# Autodesk Inventor assembly: Weapon Assembly
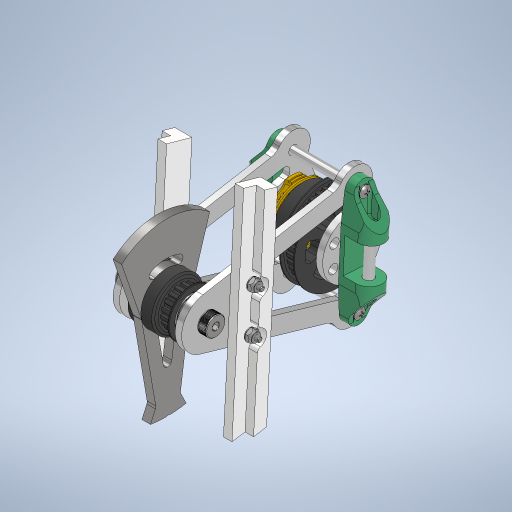
[picture p0: Inventor's stored thumbnail of the model, 512x512]
Saved by Autodesk Inventor 2023.2 (Build 272271000, 271)
## iProperties
Created: 2022-05-21
Part Number: Weapon Assembly
Document SubType Name: Assembly
Designer: Nathan Cai
Mass: 625.577 g
Surface Area: 1409.18 cm^2
Volume: 227.374 cm^3
Density: 2.75131 g/cm^3
Author: Nathan Cai
## Documents named in this file (14)
- E:\Documents\Inventor\0.3rd Lawette - V3.5\Vertical Weapon Assembly (3rd Law)\Weapon Assembly (3rd Law).iam
- E:\Documents\Inventor\0.3rd Lawette - V3.5\Standoff 1.5in.ipt
- E:\Documents\Inventor\Content Center Files\R2023\en-US\ANSI B18.6.3(27)\ANSI B18.6.3 - 6-32 UNC - 0.75(11).ipt
- E:\Documents\Inventor\Content Center Files\R2023\en-US\SAE J773b\SAE J773b - No. 6. SAE Type L. narrow.ipt
- E:\Documents\Inventor\Content Center Files\R2023\en-US\IFI 100 107(2)\IFI 100_107 - No. 6 - 32 Metal Type.ipt
- E:\Documents\Inventor\0.3rd Lawette - V3.5\Bracket.ipt
- E:\Documents\Inventor\Content Center Files\R2023\en-US\ANSI B18.6.3(27)\ANSI B18.6.3 - 6-32 UNC - 0.625(11).ipt
- E:\Documents\Inventor\0.3rd Lawette - V3.5\Vertical Weapon Assembly (3rd Law)\Legs.ipt
- E:\Documents\Inventor\0.3rd Lawette - V3.5\Vertical Weapon Assembly (3rd Law)\Frame (Motor Side).ipt
- E:\Documents\Inventor\0.3rd Lawette - V3.5\Vertical Weapon Assembly (3rd Law)\90630A121_High-Strength Steel Nylon-Insert Locknut.ipt
- E:\Documents\Inventor\0.3rd Lawette - V3.5\Vertical Weapon Assembly (3rd Law)\90807A139_Same-Size Thread Alloy Steel Shoulder Screw.ipt
- E:\Documents\Inventor\0.3rd Lawette - V3.5\Vertical Weapon Assembly (3rd Law)\Weapon (Motor-Side Pulley).iam
- E:\Documents\Inventor\0.3rd Lawette - V3.5\Vertical Weapon Assembly (3rd Law)\Weapon (Weapon-Side Pulley).iam
- E:\Documents\Inventor\0.3rd Lawette - V3.5\Standoff 2in.ipt
## Components (42 placed, 13 different names)
1. Weapon (Weapon-Side Pulley):2 [sub-assembly]
2. Weapon (Motor-Side Pulley):2 [sub-assembly] — Mate:249
3. 90807A139_Same-Size Thread Alloy Steel Shoulder Screw:2
4. 90630A121_High-Strength Steel Nylon-Insert Locknut:2
5. Frame (Motor Side):2 — Mate:245, Mate:249
6. Frame (Motor Side):3 — Mate:234, Mate:235, Mate:236, Mate:237, Mate:238, Mate:239, Mate:240, Mate:242, Mate:247
7. Legs:3 — Mate:234, Mate:235, Mate:241, Mate:243
8. Legs:2 — Mate:231, Mate:233
9. Bracket:1 — Mate:176, Flush:2, Mate:210, Mate:211, Mate:212, Mate:213, Mate:218, Mate:219, Mate:221, Mate:222, Mate:244, Mate:246, Mate:248
10. Bracket:2 — Mate:177, Flush:1, Mate:214, Mate:215, Mate:216, Mate:217, Mate:220, Mate:224, Mate:244
11. Standoff 1.5in:3 — Mate:176, Flush:2, Mate:223, Mate:225
12. Standoff 1.5in:4 — Mate:177, Flush:1
13. Cross Recessed Truss Head Machine Screw - Type I - Inch No. 6 - 32 - 3/4:29 — Mate:236, Mate:237
14. Conical Spring Washer SAE J773b (Inch) No. 6. SAE Type L. narrow:40 — Mate:240, Mate:241, Insert:47
15. Prevailing Torque Type Hex Nut - Inch (IFI) No. 6 - 32 Metal Type:24 — Insert:47
16. Cross Recessed Truss Head Machine Screw - Type I - Inch No. 6 - 32 - 3/4:30 — Mate:238, Mate:239
17. Conical Spring Washer SAE J773b (Inch) No. 6. SAE Type L. narrow:41 — Mate:242, Mate:243, Insert:48
18. Prevailing Torque Type Hex Nut - Inch (IFI) No. 6 - 32 Metal Type:25 — Insert:48
19. Standoff 2in:1 — Mate:245, Mate:246
20. Standoff 2in:2 — Mate:247, Mate:248
21. Prevailing Torque Type Hex Nut - Inch (IFI) No. 6 - 32 Metal Type:23 — Insert:46
22. Conical Spring Washer SAE J773b (Inch) No. 6. SAE Type L. narrow:39 — Mate:233, Insert:46
23. Cross Recessed Truss Head Machine Screw - Type I - Inch No. 6 - 32 - 3/4:28
24. Prevailing Torque Type Hex Nut - Inch (IFI) No. 6 - 32 Metal Type:19 — Insert:45
25. Conical Spring Washer SAE J773b (Inch) No. 6. SAE Type L. narrow:27 — Mate:231, Insert:45
26. Cross Recessed Truss Head Machine Screw - Type I - Inch No. 6 - 32 - 3/4:20
27. Cross Recessed Truss Head Machine Screw - Type I - Inch No. 6 - 32 - 5/8:8 — Insert:44
28. Conical Spring Washer SAE J773b (Inch) No. 6. SAE Type L. narrow:38 — Mate:224, Mate:225, Insert:44
29. Cross Recessed Truss Head Machine Screw - Type I - Inch No. 6 - 32 - 5/8:7 — Insert:43
30. Conical Spring Washer SAE J773b (Inch) No. 6. SAE Type L. narrow:37 — Mate:222, Mate:223, Insert:43
31. Cross Recessed Truss Head Machine Screw - Type I - Inch No. 6 - 32 - 5/8:6 — Insert:42
32. Conical Spring Washer SAE J773b (Inch) No. 6. SAE Type L. narrow:36 — Mate:220, Mate:221, Insert:42
33. Cross Recessed Truss Head Machine Screw - Type I - Inch No. 6 - 32 - 5/8:5 — Insert:41
34. Conical Spring Washer SAE J773b (Inch) No. 6. SAE Type L. narrow:35 — Mate:218, Mate:219, Insert:41
35. Cross Recessed Truss Head Machine Screw - Type I - Inch No. 6 - 32 - 3/4:27 — Insert:40
36. Conical Spring Washer SAE J773b (Inch) No. 6. SAE Type L. narrow:34 — Mate:216, Mate:217, Insert:40
37. Cross Recessed Truss Head Machine Screw - Type I - Inch No. 6 - 32 - 3/4:26 — Insert:39
38. Conical Spring Washer SAE J773b (Inch) No. 6. SAE Type L. narrow:33 — Mate:214, Mate:215, Insert:39
39. Cross Recessed Truss Head Machine Screw - Type I - Inch No. 6 - 32 - 3/4:25 — Insert:38
40. Conical Spring Washer SAE J773b (Inch) No. 6. SAE Type L. narrow:32 — Mate:212, Mate:213, Insert:38
41. Cross Recessed Truss Head Machine Screw - Type I - Inch No. 6 - 32 - 3/4:24 — Insert:37
42. Conical Spring Washer SAE J773b (Inch) No. 6. SAE Type L. narrow:31 — Mate:210, Mate:211, Insert:37
## Relationships (73: Mate 58, Insert 12, Flush 2, Symmetry 1)
- [Mate]: 90807A139_Same-Size Thread Alloy Steel Shoulder Screw:2 ↔ 90630A121_High-Strength Steel Nylon-Insert Locknut:2
- [Mate] (50.8 mm): 90807A139_Same-Size Thread Alloy Steel Shoulder Screw:2 ↔ 90630A121_High-Strength Steel Nylon-Insert Locknut:2
- [Mate]: Weapon (Weapon-Side Pulley):2 ↔ 90807A139_Same-Size Thread Alloy Steel Shoulder Screw:2
- [Mate]: 90807A139_Same-Size Thread Alloy Steel Shoulder Screw:2 ↔ Frame (Motor Side):2
- [Mate]: 90807A139_Same-Size Thread Alloy Steel Shoulder Screw:2 ↔ Frame (Motor Side):3
- [Mate]: 90807A139_Same-Size Thread Alloy Steel Shoulder Screw:2 ↔ Frame (Motor Side):3
- [Mate]: Frame (Motor Side):2 ↔ Frame (Motor Side):3
- [Mate]: Frame (Motor Side):3 ↔ Legs:3
- [Mate] (0.0254 mm): Weapon (Weapon-Side Pulley):2 ↔ Frame (Motor Side):2
- [Symmetry]: Frame (Motor Side):2 ↔ Frame (Motor Side):3
- [Mate]: Frame (Motor Side):2 ↔ Legs:2
- [Mate]: Frame (Motor Side):2 ↔ Legs:2
- [Mate]: Frame (Motor Side):2 ↔ Legs:2
- [Mate]: Weapon (Motor-Side Pulley):2 ↔ Frame (Motor Side):2
- [Mate]: Weapon (Motor-Side Pulley):2 ↔ Frame (Motor Side):2
- [Mate]: Frame (Motor Side):2 ↔ Bracket:2
- [Mate]: Frame (Motor Side):3 ↔ Bracket:1
- Mate:176: Bracket:1 ↔ Standoff 1.5in:3
- Mate:177: Bracket:2 ↔ Standoff 1.5in:4
- Flush:1: Bracket:2 ↔ Standoff 1.5in:4
- Flush:2: Bracket:1 ↔ Standoff 1.5in:3
- Mate:210: Bracket:1 ↔ Conical Spring Washer SAE J773b (Inch) No. 6. SAE Type L. narrow:31
- Mate:211: Bracket:1 ↔ Conical Spring Washer SAE J773b (Inch) No. 6. SAE Type L. narrow:31
- Mate:212: Bracket:1 ↔ Conical Spring Washer SAE J773b (Inch) No. 6. SAE Type L. narrow:32
- Mate:213: Bracket:1 ↔ Conical Spring Washer SAE J773b (Inch) No. 6. SAE Type L. narrow:32
- Insert:37: Cross Recessed Truss Head Machine Screw - Type I - Inch No. 6 - 32 - 3/4:24 ↔ Conical Spring Washer SAE J773b (Inch) No. 6. SAE Type L. narrow:31
- Insert:38: Cross Recessed Truss Head Machine Screw - Type I - Inch No. 6 - 32 - 3/4:25 ↔ Conical Spring Washer SAE J773b (Inch) No. 6. SAE Type L. narrow:32
- Mate:214: Bracket:2 ↔ Conical Spring Washer SAE J773b (Inch) No. 6. SAE Type L. narrow:33
- Mate:215: Bracket:2 ↔ Conical Spring Washer SAE J773b (Inch) No. 6. SAE Type L. narrow:33
- Mate:216: Bracket:2 ↔ Conical Spring Washer SAE J773b (Inch) No. 6. SAE Type L. narrow:34
- Mate:217: Bracket:2 ↔ Conical Spring Washer SAE J773b (Inch) No. 6. SAE Type L. narrow:34
- Insert:39: Cross Recessed Truss Head Machine Screw - Type I - Inch No. 6 - 32 - 3/4:26 ↔ Conical Spring Washer SAE J773b (Inch) No. 6. SAE Type L. narrow:33
- Insert:40: Cross Recessed Truss Head Machine Screw - Type I - Inch No. 6 - 32 - 3/4:27 ↔ Conical Spring Washer SAE J773b (Inch) No. 6. SAE Type L. narrow:34
- Mate:218: Bracket:1 ↔ Conical Spring Washer SAE J773b (Inch) No. 6. SAE Type L. narrow:35
- Mate:219: Bracket:1 ↔ Conical Spring Washer SAE J773b (Inch) No. 6. SAE Type L. narrow:35
- Mate:220: Bracket:2 ↔ Conical Spring Washer SAE J773b (Inch) No. 6. SAE Type L. narrow:36
- Mate:221: Bracket:1 ↔ Conical Spring Washer SAE J773b (Inch) No. 6. SAE Type L. narrow:36
- Insert:41: Cross Recessed Truss Head Machine Screw - Type I - Inch No. 6 - 32 - 5/8:5 ↔ Conical Spring Washer SAE J773b (Inch) No. 6. SAE Type L. narrow:35
- Insert:42: Cross Recessed Truss Head Machine Screw - Type I - Inch No. 6 - 32 - 5/8:6 ↔ Conical Spring Washer SAE J773b (Inch) No. 6. SAE Type L. narrow:36
- Mate:222: Bracket:1 ↔ Conical Spring Washer SAE J773b (Inch) No. 6. SAE Type L. narrow:37
- Mate:223: Standoff 1.5in:3 ↔ Conical Spring Washer SAE J773b (Inch) No. 6. SAE Type L. narrow:37
- Mate:224: Bracket:2 ↔ Conical Spring Washer SAE J773b (Inch) No. 6. SAE Type L. narrow:38
- Mate:225: Standoff 1.5in:3 ↔ Conical Spring Washer SAE J773b (Inch) No. 6. SAE Type L. narrow:38
- Insert:43: Cross Recessed Truss Head Machine Screw - Type I - Inch No. 6 - 32 - 5/8:7 ↔ Conical Spring Washer SAE J773b (Inch) No. 6. SAE Type L. narrow:37
- Insert:44: Cross Recessed Truss Head Machine Screw - Type I - Inch No. 6 - 32 - 5/8:8 ↔ Conical Spring Washer SAE J773b (Inch) No. 6. SAE Type L. narrow:38
- [Mate]: Frame (Motor Side):2 ↔ Cross Recessed Truss Head Machine Screw - Type I - Inch No. 6 - 32 - 3/4:20
- [Mate]: Frame (Motor Side):2 ↔ Cross Recessed Truss Head Machine Screw - Type I - Inch No. 6 - 32 - 3/4:20
- [Mate]: Frame (Motor Side):2 ↔ Cross Recessed Truss Head Machine Screw - Type I - Inch No. 6 - 32 - 3/4:28
- [Mate]: Frame (Motor Side):2 ↔ Cross Recessed Truss Head Machine Screw - Type I - Inch No. 6 - 32 - 3/4:28
- [Mate]: Frame (Motor Side):2 ↔ Conical Spring Washer SAE J773b (Inch) No. 6. SAE Type L. narrow:27
- Mate:231: Legs:2 ↔ Conical Spring Washer SAE J773b (Inch) No. 6. SAE Type L. narrow:27
- [Mate]: Frame (Motor Side):2 ↔ Conical Spring Washer SAE J773b (Inch) No. 6. SAE Type L. narrow:39
- Mate:233: Legs:2 ↔ Conical Spring Washer SAE J773b (Inch) No. 6. SAE Type L. narrow:39
- Insert:45: Prevailing Torque Type Hex Nut - Inch (IFI) No. 6 - 32 Metal Type:19 ↔ Conical Spring Washer SAE J773b (Inch) No. 6. SAE Type L. narrow:27
- Insert:46: Prevailing Torque Type Hex Nut - Inch (IFI) No. 6 - 32 Metal Type:23 ↔ Conical Spring Washer SAE J773b (Inch) No. 6. SAE Type L. narrow:39
- Mate:234: Frame (Motor Side):3 ↔ Legs:3
- Mate:235: Frame (Motor Side):3 ↔ Legs:3
- Mate:236: Frame (Motor Side):3 ↔ Cross Recessed Truss Head Machine Screw - Type I - Inch No. 6 - 32 - 3/4:29
- Mate:237: Frame (Motor Side):3 ↔ Cross Recessed Truss Head Machine Screw - Type I - Inch No. 6 - 32 - 3/4:29
- Mate:238: Frame (Motor Side):3 ↔ Cross Recessed Truss Head Machine Screw - Type I - Inch No. 6 - 32 - 3/4:30
- Mate:239: Frame (Motor Side):3 ↔ Cross Recessed Truss Head Machine Screw - Type I - Inch No. 6 - 32 - 3/4:30
- Mate:240: Frame (Motor Side):3 ↔ Conical Spring Washer SAE J773b (Inch) No. 6. SAE Type L. narrow:40
- Mate:241: Legs:3 ↔ Conical Spring Washer SAE J773b (Inch) No. 6. SAE Type L. narrow:40
- Mate:242: Frame (Motor Side):3 ↔ Conical Spring Washer SAE J773b (Inch) No. 6. SAE Type L. narrow:41
- Mate:243: Legs:3 ↔ Conical Spring Washer SAE J773b (Inch) No. 6. SAE Type L. narrow:41
- Insert:47: Conical Spring Washer SAE J773b (Inch) No. 6. SAE Type L. narrow:40 ↔ Prevailing Torque Type Hex Nut - Inch (IFI) No. 6 - 32 Metal Type:24
- Insert:48: Conical Spring Washer SAE J773b (Inch) No. 6. SAE Type L. narrow:41 ↔ Prevailing Torque Type Hex Nut - Inch (IFI) No. 6 - 32 Metal Type:25
- Mate:244 (50.8 mm): Bracket:1 ↔ Bracket:2
- Mate:245: Frame (Motor Side):2 ↔ Standoff 2in:1
- Mate:246: Bracket:1 ↔ Standoff 2in:1
- Mate:247: Frame (Motor Side):3 ↔ Standoff 2in:2
- Mate:248: Bracket:1 ↔ Standoff 2in:2
- Mate:249: Weapon (Motor-Side Pulley):2 ↔ Frame (Motor Side):2
